# Autodesk Inventor assembly: FIXT1_JAW_CAM1
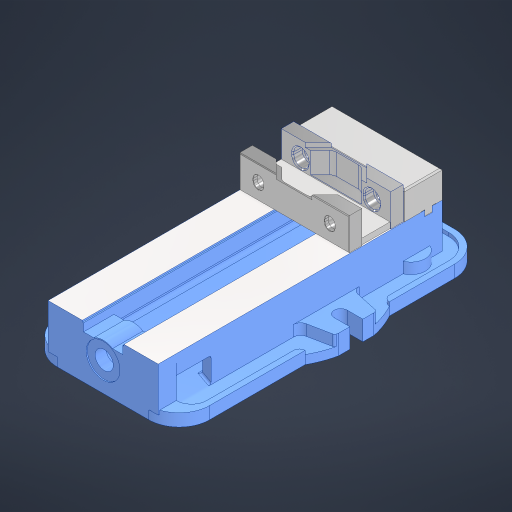
[picture p0: Inventor's stored thumbnail of the model, 512x512]
Saved by Autodesk Inventor 2024.3 (Build 283343000, 343)
## iProperties
Created: 2024-08-21
Part Number: FIXT1_JAW_CAM1
Document SubType Name: Assembly
Designer: fablabadmin
Author: fablabadmin
## Documents named in this file (7)
- C:\Users\fablabadmin\Documents\_Benjamin_S\_3dCAD\HHVerkstad\Hammer\_FIXT\_FIXT1_CAM1\_FIXT1_JAW_CAM1\FIXT1_JAW_CAM1.iam
- C:\Users\fablabadmin\Documents\_Benjamin_S\_3dCAD\_Config\KemmlerVise\OP1-KemmlerVise.iam
- C:\Users\fablabadmin\Documents\_Benjamin_S\_3dCAD\HHVerkstad\Hammer\_FIXT\_FIXT1_CAM1\JawDualSided-Aluminum 6061.ipt
- C:\Users\fablabadmin\Documents\_Benjamin_S\_3dCAD\HHVerkstad\Hammer\_FIXT\_FIXT1_CAM1\JawDualSided-Aluminum 6061MIR.ipt
- C:\Users\fablabadmin\Documents\_Benjamin_S\_3dCAD\HHVerkstad\Hammer\_FIXT\_FIXT1_CAM1\_FIXT1_JAW_CAM1\Parallel_Spacer.ipt
- C:\Users\fablabadmin\Documents\Inventor\Content Center Files\R2024\en-US\DualSidedJaw\JawDualSided-Aluminum 6061.ipt
- C:\Users\fablabadmin\Documents\_Benjamin_S\_3dCAD\_Config\_CAM_SIM\FixtureParts\parallels3mm.xlsx
## Components (7 placed, 5 different names)
1. OP1-KemmlerVise:1 [sub-assembly] — Mate:1, Mate:2, Flush:1, Mate:3, Mate:7, Mate:9, Mate:10, Flush:7, Mate:11
2. JawDualSided-Aluminum 6061:1 — Mate:1, Flush:1, Flush:2, Mate:3, Mate:6, Flush:5, Mate:13, Flush:9, Flush:10
3. JawDualSided-Aluminum 6061MIR:1 — Mate:2, Flush:2, Flush:6, Mate:8, Mate:12
4. Parallel_Spacer:1 — Mate:6, Flush:5, Flush:6, Mate:7, Mate:8
5. DualSidedJaw JawDualSided-Aluminum 6061:1 — Mate:9, Flush:7, Flush:8, Mate:11
6. DualSidedJaw JawDualSided-Aluminum 6061:2 — Mate:10, Flush:8, Mate:12
7. Parallel_Spacer:2 — Mate:13, Flush:9, Flush:10
## Relationships (19: Mate 11, Flush 8)
- Mate:1: OP1-KemmlerVise:1 ↔ JawDualSided-Aluminum 6061:1
- Mate:2: OP1-KemmlerVise:1 ↔ JawDualSided-Aluminum 6061MIR:1
- Flush:1: OP1-KemmlerVise:1 ↔ JawDualSided-Aluminum 6061:1
- Flush:2: JawDualSided-Aluminum 6061:1 ↔ JawDualSided-Aluminum 6061MIR:1
- Mate:3: OP1-KemmlerVise:1 ↔ JawDualSided-Aluminum 6061:1
- Mate:6: JawDualSided-Aluminum 6061:1 ↔ Parallel_Spacer:1
- Flush:5: JawDualSided-Aluminum 6061:1 ↔ Parallel_Spacer:1
- Flush:6: JawDualSided-Aluminum 6061MIR:1 ↔ Parallel_Spacer:1
- Mate:7: OP1-KemmlerVise:1 ↔ Parallel_Spacer:1
- Mate:8: JawDualSided-Aluminum 6061MIR:1 ↔ Parallel_Spacer:1
- Mate:9: OP1-KemmlerVise:1 ↔ DualSidedJaw JawDualSided-Aluminum 6061:1
- Mate:10: OP1-KemmlerVise:1 ↔ DualSidedJaw JawDualSided-Aluminum 6061:2
- Flush:7: OP1-KemmlerVise:1 ↔ DualSidedJaw JawDualSided-Aluminum 6061:1
- Flush:8: DualSidedJaw JawDualSided-Aluminum 6061:1 ↔ DualSidedJaw JawDualSided-Aluminum 6061:2
- Mate:11: OP1-KemmlerVise:1 ↔ DualSidedJaw JawDualSided-Aluminum 6061:1
- Mate:12: JawDualSided-Aluminum 6061MIR:1 ↔ DualSidedJaw JawDualSided-Aluminum 6061:2
- Mate:13: JawDualSided-Aluminum 6061:1 ↔ Parallel_Spacer:2
- Flush:9: JawDualSided-Aluminum 6061:1 ↔ Parallel_Spacer:2
- Flush:10 (1 mm): JawDualSided-Aluminum 6061:1 ↔ Parallel_Spacer:2
## Named parameters: PRL13 = 13 mm, PRL16 = 16 mm, PRL19 = 19 mm, PRL22 = 22 mm, PRL28 = 28 mm, PRL31 = 31 mm, PRL35 = 35 mm, PRL38 = 38 mm, PRL41 = 41 mm
